# Autodesk Inventor assembly: Chassi
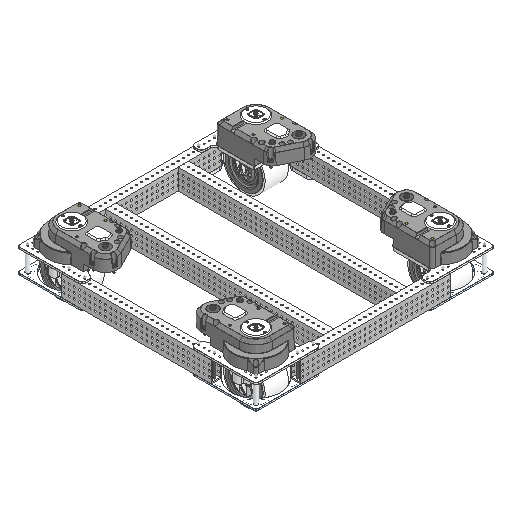
[picture p0: Inventor's stored thumbnail of the model, 512x512]
Saved by Autodesk Inventor 2025.3 (Build 293356000, 356)
## iProperties
Created: 2026-05-13
Part Number: Chassi
Document SubType Name: Assembly
Designer: djair.oliveira
Author: djair.oliveira
## Documents named in this file (5)
- C:\Users\djair.oliveira\Documents\GitHub\MT_2026\CAD\Model B\Chassi\Chassi.iam
- C:\Users\djair.oliveira\Documents\GitHub\MT_2026\CAD\Model B\MK5n, A\MK5n, A.iam
- C:\Users\djair.oliveira\Documents\GitHub\MT_2026\CAD\Model B\MK5n, B\MK5n, B.iam
- C:\Users\djair.oliveira\Documents\GitHub\MT_2026\CAD\Model B\Chassi\Forja - Base1 Chassi.ipt
- C:\Users\djair.oliveira\Documents\GitHub\MT_2026\CAD\Model B\Chassi\Forja - Base2 Chassi.ipt
## Components (10 placed, 4 different names)
1. MK5n, A:1 [sub-assembly] — Alinhado:1, Alinhado:2, Coincidente:2, Alinhado:3, Coincidente:7, Coincidente:8
2. MK5n, B:1 [sub-assembly] — Alinhado:1, Alinhado:2, Coincidente:3, Coincidente:4, Alinhado:4, Coincidente:13
3. MK5n, A:2 [sub-assembly] — Alinhado:4, Coincidente:11, Coincidente:12, Coincidente:14, Coincidente:15
4. MK5n, B:2 [sub-assembly] — Alinhado:3, Coincidente:5, Coincidente:6, Coincidente:9, Coincidente:10
5. Forja - Base1 Chassi:1 — Coincidente:2, Coincidente:3, Coincidente:4, Coincidente:19
6. Forja - Base1 Chassi:2 — Coincidente:5, Coincidente:6, Coincidente:7, Coincidente:8, Alinhado:5, Alinhado:11
7. Forja - Base1 Chassi:3 — Coincidente:9, Coincidente:10, Coincidente:11, Coincidente:12, Coincidente:18, Alinhado:9
8. Forja - Base1 Chassi:4 — Coincidente:13, Coincidente:14, Coincidente:15, Alinhado:10
9. Forja - Base2 Chassi:1 — Coincidente:18, Alinhado:9, Alinhado:10
10. Forja - Base2 Chassi:2 — Alinhado:5, Coincidente:19, Alinhado:11
## Relationships (24: Mate 16, Flush 8)
- Alinhado:1 [Flush]: MK5n, A:1 ↔ MK5n, B:1
- Alinhado:2 [Flush]: MK5n, A:1 ↔ MK5n, B:1
- Coincidente:2 [Mate]: MK5n, A:1 ↔ Forja - Base1 Chassi:1
- Coincidente:3 [Mate]: MK5n, B:1 ↔ Forja - Base1 Chassi:1
- Coincidente:4 [Mate]: MK5n, B:1 ↔ Forja - Base1 Chassi:1
- Alinhado:3 [Flush]: MK5n, A:1 ↔ MK5n, B:2
- Alinhado:4 [Flush]: MK5n, B:1 ↔ MK5n, A:2
- Coincidente:5 [Mate]: MK5n, B:2 ↔ Forja - Base1 Chassi:2
- Coincidente:6 [Mate]: MK5n, B:2 ↔ Forja - Base1 Chassi:2
- Coincidente:7 [Mate]: MK5n, A:1 ↔ Forja - Base1 Chassi:2
- Coincidente:8 [Mate]: MK5n, A:1 ↔ Forja - Base1 Chassi:2
- Coincidente:9 [Mate]: MK5n, B:2 ↔ Forja - Base1 Chassi:3
- Coincidente:10 [Mate]: MK5n, B:2 ↔ Forja - Base1 Chassi:3
- Coincidente:11 [Mate]: MK5n, A:2 ↔ Forja - Base1 Chassi:3
- Coincidente:12 [Mate]: MK5n, A:2 ↔ Forja - Base1 Chassi:3
- Coincidente:13 [Mate]: MK5n, B:1 ↔ Forja - Base1 Chassi:4
- Coincidente:14 [Mate]: MK5n, A:2 ↔ Forja - Base1 Chassi:4
- Coincidente:15 [Mate]: MK5n, A:2 ↔ Forja - Base1 Chassi:4
- Alinhado:5 [Flush]: Forja - Base1 Chassi:2 ↔ Forja - Base2 Chassi:2
- Coincidente:18 [Mate]: Forja - Base1 Chassi:3 ↔ Forja - Base2 Chassi:1
- Alinhado:9 [Flush]: Forja - Base1 Chassi:3 ↔ Forja - Base2 Chassi:1
- Alinhado:10 [Flush] (190.5 mm): Forja - Base1 Chassi:4 ↔ Forja - Base2 Chassi:1
- Coincidente:19 [Mate]: Forja - Base1 Chassi:1 ↔ Forja - Base2 Chassi:2
- Alinhado:11 [Flush] (190.5 mm): Forja - Base1 Chassi:2 ↔ Forja - Base2 Chassi:2
